# Autodesk Inventor assembly: fabrication model end cap left
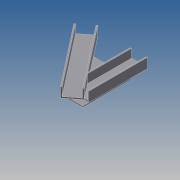
[picture p0: Inventor's stored thumbnail of the model, 180x180]
Saved by Autodesk Inventor 2014 SP1 (Build 180222100, 222)
## iProperties
Created: 2015-02-10
Part Number: fabrication model end cap left
Document SubType Name: Assembly
Designer: degan
Author: degan
## Documents named in this file (5)
- C:\Users\Dave\Desktop\hera-cad\endcaps\fabrication model end cap left.iam
- C:\Users\Dave\Desktop\hera-cad\endcaps\ring support left.ipt
- C:\Users\Dave\Desktop\hera-cad\endcaps\angle channel.ipt
- C:\Users\Dave\Desktop\hera-cad\endcaps\Horizontal channel left.ipt
- C:\Users\Dave\Desktop\hera-cad\endcaps\side plate.ipt
## Components (4 placed, 4 different names)
1. ring support left:1 — Mate:5, Mate:6
2. angle channel:1 — Mate:1, Flush:1, Flush:2, Mate:4, Flush:4, Mate:6
3. Horizontal channel left:1 — Mate:1, Flush:1, Mate:2, Angle:1, Flush:5
4. side plate:1 — Mate:4, Flush:4, Flush:5, Mate:5
## Relationships (10: Mate 5, Flush 4, Angle 1)
- Mate:1: angle channel:1 ↔ Horizontal channel left:1
- Flush:1: angle channel:1 ↔ Horizontal channel left:1
- Mate:2: Horizontal channel left:1
- Angle:1 (90 deg): Horizontal channel left:1
- Flush:2: angle channel:1
- Mate:4: angle channel:1 ↔ side plate:1
- Flush:4: angle channel:1 ↔ side plate:1
- Flush:5: Horizontal channel left:1 ↔ side plate:1
- Mate:5: ring support left:1 ↔ side plate:1
- Mate:6: ring support left:1 ↔ angle channel:1
